# Autodesk Inventor assembly: Spring Assembly
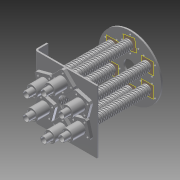
[picture p0: Inventor's stored thumbnail of the model, 180x180]
Saved by Autodesk Inventor 2014 (Build 180170000, 170)
## iProperties
Created: 2014-01-12
Part Number: Spring Assembly
Document SubType Name: Assembly
Designer: Andrew Toennies
Author: Andrew Toennies
## Documents named in this file (6)
- C:\Users\Andrew Toennies\Documents\GitHub\2014buildCAD\Shooter\Launching Mechanism\Spring Assembly.iam
- C:\Users\Andrew Toennies\Documents\GitHub\2014buildCAD\Shooter\Launching Mechanism\Plate (Front).ipt
- C:\Users\Andrew Toennies\Documents\GitHub\2014buildCAD\Shooter\Launching Mechanism\Spring 9657K213.ipt
- C:\Users\Andrew Toennies\Documents\GitHub\2014buildCAD\Shooter\Launching Mechanism\Shaft (0.500 Aluminum.ipt
- C:\Users\Andrew Toennies\Documents\GitHub\2014buildCAD\Shooter\Launching Mechanism\Plate 2 (Back).ipt
- C:\Users\Andrew Toennies\Documents\GitHub\2014buildCAD\Shooter\Launching Mechanism\Linear Bearing 6483K630.ipt
## Components (20 placed, 5 different names)
1. Plate (Front):1 — Mate:1, Mate:2, Mate:3, Mate:4, Mate:5, Mate:6, Flush:1, Flush:2, Flush:3, Flush:4, Flush:5, Flush:6, Flush:7, Mate:7, Mate:8, Flush:8, Mate:9, Flush:9, Mate:10, Flush:10, Mate:11, Flush:11, Mate:12, Flush:12
2. Shaft (0.500 Aluminum:1 — Mate:11, Flush:11, Mate:14
3. Shaft (0.500 Aluminum:2 — Flush:7, Mate:7
4. Shaft (0.500 Aluminum:3 — Mate:10, Flush:10
5. Shaft (0.500 Aluminum:4 — Mate:12, Flush:12
6. Shaft (0.500 Aluminum:5 — Mate:9, Flush:9, Mate:16
7. Shaft (0.500 Aluminum:6 — Mate:8, Flush:8, Mate:13
8. Plate 2 (Back):1 — Mate:13, Mate:14, Mate:15, Mate:16, Mate:17, Mate:18, Mate:19, Mate:20, Mate:21, Mate:22, Mate:23, Mate:24, Mate:25, Mate:26, Mate:27, Mate:28, Mate:29, Mate:30, Mate:31, Mate:32, Mate:33, Mate:34
9. Linear Bearing 6483K630:1 — Mate:26, Mate:27, Mate:28
10. Linear Bearing 6483K630:2 — Mate:32, Mate:33, Mate:34
11. Linear Bearing 6483K630:3 — Mate:23, Mate:24, Mate:25
12. Linear Bearing 6483K630:4 — Mate:29, Mate:30, Mate:31
13. Linear Bearing 6483K630:5 — Mate:20, Mate:21, Mate:22
14. Linear Bearing 6483K630:6 — Mate:17, Mate:18, Mate:19
15. Spring 9657K213:1 — Mate:4, Flush:5
16. Spring 9657K213:2 — Mate:6, Flush:4
17. Spring 9657K213:3 — Mate:1, Flush:1
18. Spring 9657K213:4 — Mate:3, Flush:2
19. Spring 9657K213:5 — Mate:5, Flush:6
20. Spring 9657K213:6 — Mate:2, Flush:3, Mate:15
## Relationships (46: Mate 34, Flush 12)
- Mate:1: Plate (Front):1 ↔ Spring 9657K213:3
- Mate:2: Plate (Front):1 ↔ Spring 9657K213:6
- Mate:3: Plate (Front):1 ↔ Spring 9657K213:4
- Mate:4: Plate (Front):1 ↔ Spring 9657K213:1
- Mate:5: Plate (Front):1 ↔ Spring 9657K213:5
- Mate:6: Plate (Front):1 ↔ Spring 9657K213:2
- Flush:1: Plate (Front):1 ↔ Spring 9657K213:3
- Flush:2: Plate (Front):1 ↔ Spring 9657K213:4
- Flush:3: Plate (Front):1 ↔ Spring 9657K213:6
- Flush:4: Plate (Front):1 ↔ Spring 9657K213:2
- Flush:5: Plate (Front):1 ↔ Spring 9657K213:1
- Flush:6: Plate (Front):1 ↔ Spring 9657K213:5
- Flush:7: Plate (Front):1 ↔ Shaft (0.500 Aluminum:2
- Mate:7: Plate (Front):1 ↔ Shaft (0.500 Aluminum:2
- Mate:8: Plate (Front):1 ↔ Shaft (0.500 Aluminum:6
- Flush:8: Plate (Front):1 ↔ Shaft (0.500 Aluminum:6
- Mate:9: Plate (Front):1 ↔ Shaft (0.500 Aluminum:5
- Flush:9: Plate (Front):1 ↔ Shaft (0.500 Aluminum:5
- Mate:10: Plate (Front):1 ↔ Shaft (0.500 Aluminum:3
- Flush:10: Plate (Front):1 ↔ Shaft (0.500 Aluminum:3
- Mate:11: Plate (Front):1 ↔ Shaft (0.500 Aluminum:1
- Flush:11: Plate (Front):1 ↔ Shaft (0.500 Aluminum:1
- Mate:12: Plate (Front):1 ↔ Shaft (0.500 Aluminum:4
- Flush:12: Plate (Front):1 ↔ Shaft (0.500 Aluminum:4
- Mate:13: Shaft (0.500 Aluminum:6 ↔ Plate 2 (Back):1
- Mate:14: Shaft (0.500 Aluminum:1 ↔ Plate 2 (Back):1
- Mate:15: Plate 2 (Back):1 ↔ Spring 9657K213:6
- Mate:16: Shaft (0.500 Aluminum:5 ↔ Plate 2 (Back):1
- Mate:17: Plate 2 (Back):1 ↔ Linear Bearing 6483K630:6
- Mate:18: Plate 2 (Back):1 ↔ Linear Bearing 6483K630:6
- Mate:19: Plate 2 (Back):1 ↔ Linear Bearing 6483K630:6
- Mate:20: Plate 2 (Back):1 ↔ Linear Bearing 6483K630:5
- Mate:21: Plate 2 (Back):1 ↔ Linear Bearing 6483K630:5
- Mate:22: Plate 2 (Back):1 ↔ Linear Bearing 6483K630:5
- Mate:23: Plate 2 (Back):1 ↔ Linear Bearing 6483K630:3
- Mate:24: Plate 2 (Back):1 ↔ Linear Bearing 6483K630:3
- Mate:25: Plate 2 (Back):1 ↔ Linear Bearing 6483K630:3
- Mate:26: Plate 2 (Back):1 ↔ Linear Bearing 6483K630:1
- Mate:27: Plate 2 (Back):1 ↔ Linear Bearing 6483K630:1
- Mate:28: Plate 2 (Back):1 ↔ Linear Bearing 6483K630:1
- Mate:29: Plate 2 (Back):1 ↔ Linear Bearing 6483K630:4
- Mate:30: Plate 2 (Back):1 ↔ Linear Bearing 6483K630:4
- Mate:31: Plate 2 (Back):1 ↔ Linear Bearing 6483K630:4
- Mate:32: Plate 2 (Back):1 ↔ Linear Bearing 6483K630:2
- Mate:33: Plate 2 (Back):1 ↔ Linear Bearing 6483K630:2
- Mate:34: Plate 2 (Back):1 ↔ Linear Bearing 6483K630:2
